# Autodesk Inventor assembly: 3FlexWheel
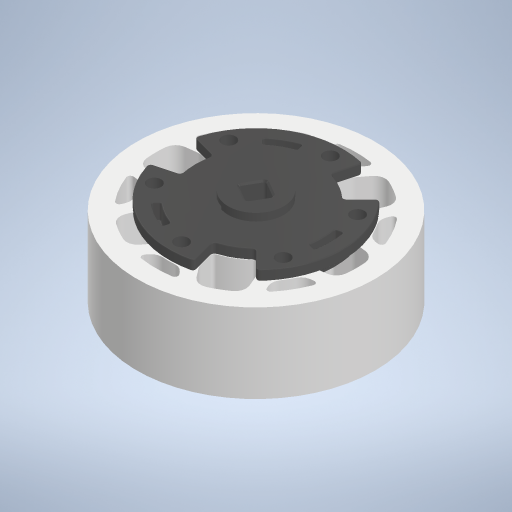
[picture p0: Inventor's stored thumbnail of the model, 512x512]
Saved by Autodesk Inventor 2023 (Build 270158000, 158)
## iProperties
Created: 2022-09-10
Part Number: 3FlexWheel
Document SubType Name: Assembly
Designer: alex
Author: alex
## Documents named in this file (5)
- C:\Users\alex\Documents\GitHub\4067X_spin_up_cad\Library\3FlexWheel.iam
- C:\Users\alex\Documents\GitHub\4067X_spin_up_cad\Library\Motion\Wheels\Flex Wheels\3.000 Flex Wheel\3.000 30A 1.000.ipt
- C:\Users\alex\Documents\GitHub\4067X_spin_up_cad\Library\Motion\Wheels\Flex Wheels\3.000 Flex Wheel.ipt
- C:\Users\alex\Documents\GitHub\4067X_spin_up_cad\Library\Motion\Wheels\Flex Wheels\VersaHub.ipt
- C:\Users\alex\Documents\GitHub\4067X_spin_up_cad\Library\Motion\Wheels\Flex Wheels\VersaHex Adapters .250.ipt
## Components (5 placed, 3 different names)
1. 3.000 30A 1.000:1 — Mate:1, Mate:2, Mate:3, Mate:10, Mate:11, Mate:12
2. VersaHub:1 — Mate:1, Mate:2, Mate:3, Mate:4, Mate:5, Mate:6
3. VersaHex Adapters .250:1 — Mate:4, Mate:5, Mate:6
4. VersaHub:2 — Mate:10, Mate:11, Mate:12
5. VersaHex Adapters .250:2
## Relationships (12: Mate 12)
- Mate:1: 3.000 30A 1.000:1 ↔ VersaHub:1
- Mate:2: 3.000 30A 1.000:1 ↔ VersaHub:1
- Mate:3: 3.000 30A 1.000:1 ↔ VersaHub:1
- Mate:4: VersaHub:1 ↔ VersaHex Adapters .250:1
- Mate:5: VersaHub:1 ↔ VersaHex Adapters .250:1
- Mate:6: VersaHub:1 ↔ VersaHex Adapters .250:1
- [Mate]: VersaHub:2 ↔ VersaHex Adapters .250:2
- [Mate]: VersaHub:2 ↔ VersaHex Adapters .250:2
- [Mate]: VersaHub:2 ↔ VersaHex Adapters .250:2
- Mate:10: 3.000 30A 1.000:1 ↔ VersaHub:2
- Mate:11: 3.000 30A 1.000:1 ↔ VersaHub:2
- Mate:12: 3.000 30A 1.000:1 ↔ VersaHub:2
## Named parameters: d6_d3 = 0 mm, d7_d4 = 0 mm, d8_d5 = 0 mm
